# Autodesk Inventor assembly: Assembly2
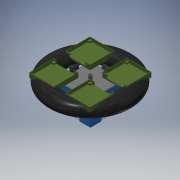
[picture p0: Inventor's stored thumbnail of the model, 180x180]
Saved by Autodesk Inventor 2017 (Build 210142000, 142)
## iProperties
Created: 2017-01-20
Part Number: Assembly2
Document SubType Name: Assembly
Designer: jbui8
Author: jbui8
## Documents named in this file (3)
- C:\Users\jbui8\Google Drive\Undergraduate\Undergraduate Research\Static PV Electrolyzer\CAD Files\Floating Reactor Design\Reactor Parts\Assembly Parts\Assembly2.iam
- C:\Users\jbui8\Google Drive\Undergraduate\Undergraduate Research\Static PV Electrolyzer\CAD Files\Floating Reactor Design\Reactor Parts\Assembly Parts\Subassembly1.iam
- C:\Users\jbui8\Google Drive\Undergraduate\Undergraduate Research\Static PV Electrolyzer\CAD Files\Floating Reactor Design\Reactor Parts\Assembly Parts\Subassembly2.iam
## Components (2 placed, 2 different names)
1. Subassembly1:1 [sub-assembly] — Mate:1, Mate:2
2. Subassembly2:1 [sub-assembly] — Mate:1, Mate:2
## Relationships (2: Mate 2)
- Mate:1: Subassembly1:1 ↔ Subassembly2:1
- Mate:2: Subassembly1:1 ↔ Subassembly2:1
